# Autodesk Inventor assembly: oswietlacz
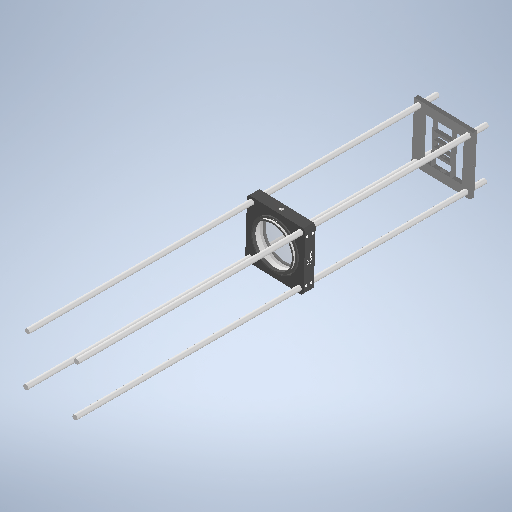
[picture p0: Inventor's stored thumbnail of the model, 512x512]
Saved by Autodesk Inventor 2025.1 (Build 291241020, 241B)
## iProperties
Created: 2024-10-13
Part Number: oswietlacz
Document SubType Name: Assembly
Designer: zychlix
Author: zychlix
## Documents named in this file (6)
- C:\Users\zychlix\Fotolitografia\oswietlacz.iam
- C:\Users\zychlix\Fotolitografia\rod.ipt
- C:\Users\zychlix\Fotolitografia\LCP09-Solidworks.ipt
- C:\Users\zychlix\Fotolitografia\LA1979-A-Solidworks.ipt
- C:\Users\zychlix\Fotolitografia\SM2L05-Solidworks.ipt
- C:\Users\zychlix\Fotolitografia\led_holder.ipt
## Components (8 placed, 5 different names)
1. rod:1 — Zestawiające:4, Równoległe:2, Zestawiające:7
2. rod:2 — Zestawiające:3, Równoległe:1, Równoległe:2
3. rod:3 — Zestawiające:1, Równoległe:1, Równoległe:3, Zestawiające:8
4. rod:4 — Zestawiające:2, Równoległe:3
5. LCP09-Solidworks:1 — Zestawiające:1, Zestawiające:2, Zestawiające:3, Zestawiające:4, Zestawiające:5, Równoległe:4, Zestawiające:6, Równoległe:5
6. LA1979-A-Solidworks:1 — Zestawiające:5, Równoległe:4
7. SM2L05-Solidworks:1 — Zestawiające:6, Równoległe:5
8. led_holder:1 — Zestawiające:7, Zestawiające:8
## Relationships (13: Mate 8, Flush 5)
- Zestawiające:1 [Mate]: rod:3 ↔ LCP09-Solidworks:1
- Zestawiające:2 [Mate]: rod:4 ↔ LCP09-Solidworks:1
- Zestawiające:3 [Mate]: rod:2 ↔ LCP09-Solidworks:1
- Zestawiające:4 [Mate]: rod:1 ↔ LCP09-Solidworks:1
- Równoległe:1 [Flush]: rod:2 ↔ rod:3
- Równoległe:2 [Flush]: rod:1 ↔ rod:2
- Równoległe:3 [Flush]: rod:3 ↔ rod:4
- Zestawiające:5 [Mate]: LCP09-Solidworks:1 ↔ LA1979-A-Solidworks:1
- Równoległe:4 [Flush] (-3 mm): LCP09-Solidworks:1 ↔ LA1979-A-Solidworks:1
- Zestawiające:6 [Mate]: LCP09-Solidworks:1 ↔ SM2L05-Solidworks:1
- Zestawiające:7 [Mate]: rod:1 ↔ led_holder:1
- Zestawiające:8 [Mate]: rod:3 ↔ led_holder:1
- Równoległe:5 [Flush]: LCP09-Solidworks:1 ↔ SM2L05-Solidworks:1
